# Autodesk Inventor assembly: Weapon Assembly
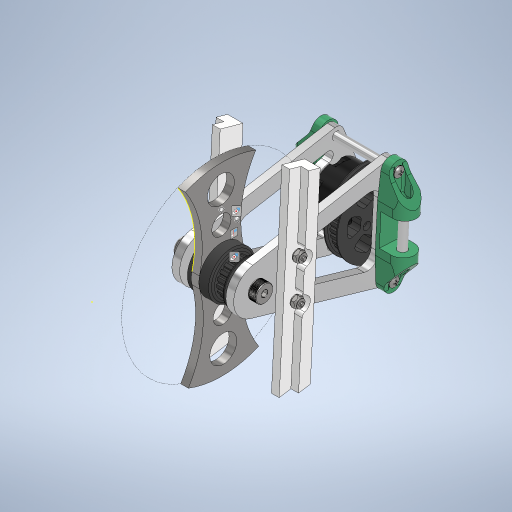
[picture p0: Inventor's stored thumbnail of the model, 512x512]
Saved by Autodesk Inventor 2023.2 (Build 272271000, 271)
## iProperties
Created: 2022-05-21
Part Number: Weapon Assembly
Document SubType Name: Assembly
Designer: Nathan Cai
Mass: 728.967 g
Surface Area: 1305.35 cm^2
Volume: 220.476 cm^3
Density: 3.30633 g/cm^3
Author: Nathan Cai
## Documents named in this file (14)
- E:\Documents\Inventor\0.3rd Lawette - V3.5\Vertical Weapon Assembly (3rd Law)\Weapon Assembly (Vert A).iam
- E:\Documents\Inventor\0.3rd Lawette - V3.5\Standoff 1.5in.ipt
- E:\Documents\Inventor\Content Center Files\R2023\en-US\ANSI B18.6.3(27)\ANSI B18.6.3 - 6-32 UNC - 0.75(11).ipt
- E:\Documents\Inventor\Content Center Files\R2023\en-US\SAE J773b\SAE J773b - No. 6. SAE Type L. narrow.ipt
- E:\Documents\Inventor\Content Center Files\R2023\en-US\IFI 100 107(2)\IFI 100_107 - No. 6 - 32 Metal Type.ipt
- E:\Documents\Inventor\0.3rd Lawette - V3.5\Bracket.ipt
- E:\Documents\Inventor\Content Center Files\R2023\en-US\ANSI B18.6.3(27)\ANSI B18.6.3 - 6-32 UNC - 0.625(11).ipt
- E:\Documents\Inventor\0.3rd Lawette - V3.5\Vertical Weapon Assembly (3rd Law)\Legs.ipt
- E:\Documents\Inventor\0.3rd Lawette - V3.5\Vertical Weapon Assembly (3rd Law)\Frame (Clear Side).ipt
- E:\Documents\Inventor\0.3rd Lawette - V3.5\Vertical Weapon Assembly (3rd Law)\Frame (Motor Side).ipt
- E:\Documents\Inventor\0.3rd Lawette - V3.5\Vertical Weapon Assembly (3rd Law)\90630A121_High-Strength Steel Nylon-Insert Locknut.ipt
- E:\Documents\Inventor\0.3rd Lawette - V3.5\Vertical Weapon Assembly (3rd Law)\90807A139_Same-Size Thread Alloy Steel Shoulder Screw.ipt
- E:\Documents\Inventor\0.3rd Lawette - V3.5\Vertical Weapon Assembly (3rd Law)\Weapon (Motor-Side Pulley).iam
- E:\Documents\Inventor\0.3rd Lawette - V3.5\Vertical Weapon Assembly (3rd Law)\Weapon (Weapon-Side Pulley).iam
## Components (42 placed, 13 different names)
1. Weapon (Weapon-Side Pulley):2 [sub-assembly]
2. Weapon (Motor-Side Pulley):2 [sub-assembly]
3. 90807A139_Same-Size Thread Alloy Steel Shoulder Screw:2
4. 90630A121_High-Strength Steel Nylon-Insert Locknut:2
5. Frame (Motor Side):2
6. Frame (Clear Side):2
7. Legs:3
8. Legs:2 — Mate:231, Mate:233
9. Bracket:1 — Mate:174, Mate:175, Mate:176, Flush:2, Mate:210, Mate:211, Mate:212, Mate:213, Mate:218, Mate:219, Mate:221, Mate:222
10. Bracket:2 — Mate:171, Mate:172, Mate:177, Flush:1, Mate:214, Mate:215, Mate:216, Mate:217, Mate:220, Mate:224
11. Standoff 1.5in:1 — Mate:171, Mate:174
12. Standoff 1.5in:2 — Mate:172, Mate:175
13. Standoff 1.5in:3 — Mate:176, Flush:2, Mate:223, Mate:225
14. Standoff 1.5in:4 — Mate:177, Flush:1
15. Prevailing Torque Type Hex Nut - Inch (IFI) No. 6 - 32 Metal Type:23 — Insert:46
16. Conical Spring Washer SAE J773b (Inch) No. 6. SAE Type L. narrow:39 — Mate:233, Insert:46
17. Cross Recessed Truss Head Machine Screw - Type I - Inch No. 6 - 32 - 3/4:28
18. Prevailing Torque Type Hex Nut - Inch (IFI) No. 6 - 32 Metal Type:19 — Insert:45
19. Conical Spring Washer SAE J773b (Inch) No. 6. SAE Type L. narrow:27 — Mate:231, Insert:45
20. Cross Recessed Truss Head Machine Screw - Type I - Inch No. 6 - 32 - 3/4:20
21. Cross Recessed Truss Head Machine Screw - Type I - Inch No. 6 - 32 - 5/8:8 — Insert:44
22. Conical Spring Washer SAE J773b (Inch) No. 6. SAE Type L. narrow:38 — Mate:224, Mate:225, Insert:44
23. Cross Recessed Truss Head Machine Screw - Type I - Inch No. 6 - 32 - 5/8:7 — Insert:43
24. Conical Spring Washer SAE J773b (Inch) No. 6. SAE Type L. narrow:37 — Mate:222, Mate:223, Insert:43
25. Cross Recessed Truss Head Machine Screw - Type I - Inch No. 6 - 32 - 5/8:6 — Insert:42
26. Conical Spring Washer SAE J773b (Inch) No. 6. SAE Type L. narrow:36 — Mate:220, Mate:221, Insert:42
27. Cross Recessed Truss Head Machine Screw - Type I - Inch No. 6 - 32 - 5/8:5 — Insert:41
28. Conical Spring Washer SAE J773b (Inch) No. 6. SAE Type L. narrow:35 — Mate:218, Mate:219, Insert:41
29. Cross Recessed Truss Head Machine Screw - Type I - Inch No. 6 - 32 - 3/4:27 — Insert:40
30. Conical Spring Washer SAE J773b (Inch) No. 6. SAE Type L. narrow:34 — Mate:216, Mate:217, Insert:40
31. Cross Recessed Truss Head Machine Screw - Type I - Inch No. 6 - 32 - 3/4:26 — Insert:39
32. Conical Spring Washer SAE J773b (Inch) No. 6. SAE Type L. narrow:33 — Mate:214, Mate:215, Insert:39
33. Cross Recessed Truss Head Machine Screw - Type I - Inch No. 6 - 32 - 3/4:25 — Insert:38
34. Conical Spring Washer SAE J773b (Inch) No. 6. SAE Type L. narrow:32 — Mate:212, Mate:213, Insert:38
35. Cross Recessed Truss Head Machine Screw - Type I - Inch No. 6 - 32 - 3/4:24 — Insert:37
36. Conical Spring Washer SAE J773b (Inch) No. 6. SAE Type L. narrow:31 — Mate:210, Mate:211, Insert:37
37. Prevailing Torque Type Hex Nut - Inch (IFI) No. 6 - 32 Metal Type:22 — Insert:36
38. Conical Spring Washer SAE J773b (Inch) No. 6. SAE Type L. narrow:30 — Insert:36
39. Cross Recessed Truss Head Machine Screw - Type I - Inch No. 6 - 32 - 3/4:23
40. Prevailing Torque Type Hex Nut - Inch (IFI) No. 6 - 32 Metal Type:21 — Insert:35
41. Conical Spring Washer SAE J773b (Inch) No. 6. SAE Type L. narrow:29 — Insert:35
42. Cross Recessed Truss Head Machine Screw - Type I - Inch No. 6 - 32 - 3/4:22
## Relationships (77: Mate 62, Insert 12, Flush 2, Symmetry 1)
- [Mate]: 90807A139_Same-Size Thread Alloy Steel Shoulder Screw:2 ↔ 90630A121_High-Strength Steel Nylon-Insert Locknut:2
- [Mate] (50.8 mm): 90807A139_Same-Size Thread Alloy Steel Shoulder Screw:2 ↔ 90630A121_High-Strength Steel Nylon-Insert Locknut:2
- [Mate]: Weapon (Weapon-Side Pulley):2 ↔ 90807A139_Same-Size Thread Alloy Steel Shoulder Screw:2
- [Mate]: 90807A139_Same-Size Thread Alloy Steel Shoulder Screw:2 ↔ Frame (Motor Side):2
- [Mate]: 90807A139_Same-Size Thread Alloy Steel Shoulder Screw:2 ↔ Frame (Clear Side):2
- [Mate]: 90807A139_Same-Size Thread Alloy Steel Shoulder Screw:2 ↔ Frame (Clear Side):2
- [Mate]: Frame (Motor Side):2 ↔ Frame (Clear Side):2
- [Mate]: Frame (Motor Side):2 ↔ Standoff 1.5in:1
- [Mate]: Frame (Motor Side):2 ↔ Standoff 1.5in:2
- [Mate]: Frame (Motor Side):2 ↔ Standoff 1.5in:1
- [Mate]: Frame (Motor Side):2 ↔ Standoff 1.5in:2
- [Mate]: Frame (Clear Side):2 ↔ Legs:3
- [Mate]: Frame (Clear Side):2 ↔ Legs:3
- [Mate]: Frame (Clear Side):2 ↔ Legs:3
- [Mate]: Frame (Clear Side):2 ↔ Standoff 1.5in:1
- [Mate] (0.0254 mm): Weapon (Weapon-Side Pulley):2 ↔ Frame (Motor Side):2
- [Symmetry]: Frame (Motor Side):2 ↔ Frame (Clear Side):2
- [Mate]: Frame (Motor Side):2 ↔ Legs:2
- [Mate]: Frame (Motor Side):2 ↔ Legs:2
- [Mate]: Frame (Motor Side):2 ↔ Legs:2
- [Mate]: Weapon (Motor-Side Pulley):2 ↔ Frame (Motor Side):2
- [Mate]: Weapon (Motor-Side Pulley):2 ↔ Frame (Motor Side):2
- [Mate]: Weapon (Motor-Side Pulley):2 ↔ Frame (Motor Side):2
- [Mate]: Frame (Motor Side):2 ↔ Bracket:2
- Mate:171: Bracket:2 ↔ Standoff 1.5in:1
- Mate:172: Bracket:2 ↔ Standoff 1.5in:2
- [Mate]: Frame (Clear Side):2 ↔ Bracket:1
- Mate:174: Bracket:1 ↔ Standoff 1.5in:1
- Mate:175: Bracket:1 ↔ Standoff 1.5in:2
- Mate:176: Bracket:1 ↔ Standoff 1.5in:3
- Mate:177: Bracket:2 ↔ Standoff 1.5in:4
- Flush:1: Bracket:2 ↔ Standoff 1.5in:4
- Flush:2: Bracket:1 ↔ Standoff 1.5in:3
- [Mate]: Frame (Clear Side):2 ↔ Cross Recessed Truss Head Machine Screw - Type I - Inch No. 6 - 32 - 3/4:22
- [Mate]: Frame (Clear Side):2 ↔ Cross Recessed Truss Head Machine Screw - Type I - Inch No. 6 - 32 - 3/4:22
- [Mate]: Frame (Clear Side):2 ↔ Cross Recessed Truss Head Machine Screw - Type I - Inch No. 6 - 32 - 3/4:23
- [Mate]: Frame (Clear Side):2 ↔ Cross Recessed Truss Head Machine Screw - Type I - Inch No. 6 - 32 - 3/4:23
- [Mate]: Frame (Clear Side):2 ↔ Conical Spring Washer SAE J773b (Inch) No. 6. SAE Type L. narrow:29
- [Mate]: Legs:3 ↔ Conical Spring Washer SAE J773b (Inch) No. 6. SAE Type L. narrow:29
- [Mate]: Frame (Clear Side):2 ↔ Conical Spring Washer SAE J773b (Inch) No. 6. SAE Type L. narrow:30
- [Mate]: Legs:3 ↔ Conical Spring Washer SAE J773b (Inch) No. 6. SAE Type L. narrow:30
- Insert:35: Prevailing Torque Type Hex Nut - Inch (IFI) No. 6 - 32 Metal Type:21 ↔ Conical Spring Washer SAE J773b (Inch) No. 6. SAE Type L. narrow:29
- Insert:36: Prevailing Torque Type Hex Nut - Inch (IFI) No. 6 - 32 Metal Type:22 ↔ Conical Spring Washer SAE J773b (Inch) No. 6. SAE Type L. narrow:30
- Mate:210: Bracket:1 ↔ Conical Spring Washer SAE J773b (Inch) No. 6. SAE Type L. narrow:31
- Mate:211: Bracket:1 ↔ Conical Spring Washer SAE J773b (Inch) No. 6. SAE Type L. narrow:31
- Mate:212: Bracket:1 ↔ Conical Spring Washer SAE J773b (Inch) No. 6. SAE Type L. narrow:32
- Mate:213: Bracket:1 ↔ Conical Spring Washer SAE J773b (Inch) No. 6. SAE Type L. narrow:32
- Insert:37: Cross Recessed Truss Head Machine Screw - Type I - Inch No. 6 - 32 - 3/4:24 ↔ Conical Spring Washer SAE J773b (Inch) No. 6. SAE Type L. narrow:31
- Insert:38: Cross Recessed Truss Head Machine Screw - Type I - Inch No. 6 - 32 - 3/4:25 ↔ Conical Spring Washer SAE J773b (Inch) No. 6. SAE Type L. narrow:32
- Mate:214: Bracket:2 ↔ Conical Spring Washer SAE J773b (Inch) No. 6. SAE Type L. narrow:33
- Mate:215: Bracket:2 ↔ Conical Spring Washer SAE J773b (Inch) No. 6. SAE Type L. narrow:33
- Mate:216: Bracket:2 ↔ Conical Spring Washer SAE J773b (Inch) No. 6. SAE Type L. narrow:34
- Mate:217: Bracket:2 ↔ Conical Spring Washer SAE J773b (Inch) No. 6. SAE Type L. narrow:34
- Insert:39: Cross Recessed Truss Head Machine Screw - Type I - Inch No. 6 - 32 - 3/4:26 ↔ Conical Spring Washer SAE J773b (Inch) No. 6. SAE Type L. narrow:33
- Insert:40: Cross Recessed Truss Head Machine Screw - Type I - Inch No. 6 - 32 - 3/4:27 ↔ Conical Spring Washer SAE J773b (Inch) No. 6. SAE Type L. narrow:34
- Mate:218: Bracket:1 ↔ Conical Spring Washer SAE J773b (Inch) No. 6. SAE Type L. narrow:35
- Mate:219: Bracket:1 ↔ Conical Spring Washer SAE J773b (Inch) No. 6. SAE Type L. narrow:35
- Mate:220: Bracket:2 ↔ Conical Spring Washer SAE J773b (Inch) No. 6. SAE Type L. narrow:36
- Mate:221: Bracket:1 ↔ Conical Spring Washer SAE J773b (Inch) No. 6. SAE Type L. narrow:36
- Insert:41: Cross Recessed Truss Head Machine Screw - Type I - Inch No. 6 - 32 - 5/8:5 ↔ Conical Spring Washer SAE J773b (Inch) No. 6. SAE Type L. narrow:35
- Insert:42: Cross Recessed Truss Head Machine Screw - Type I - Inch No. 6 - 32 - 5/8:6 ↔ Conical Spring Washer SAE J773b (Inch) No. 6. SAE Type L. narrow:36
- Mate:222: Bracket:1 ↔ Conical Spring Washer SAE J773b (Inch) No. 6. SAE Type L. narrow:37
- Mate:223: Standoff 1.5in:3 ↔ Conical Spring Washer SAE J773b (Inch) No. 6. SAE Type L. narrow:37
- Mate:224: Bracket:2 ↔ Conical Spring Washer SAE J773b (Inch) No. 6. SAE Type L. narrow:38
- Mate:225: Standoff 1.5in:3 ↔ Conical Spring Washer SAE J773b (Inch) No. 6. SAE Type L. narrow:38
- Insert:43: Cross Recessed Truss Head Machine Screw - Type I - Inch No. 6 - 32 - 5/8:7 ↔ Conical Spring Washer SAE J773b (Inch) No. 6. SAE Type L. narrow:37
- Insert:44: Cross Recessed Truss Head Machine Screw - Type I - Inch No. 6 - 32 - 5/8:8 ↔ Conical Spring Washer SAE J773b (Inch) No. 6. SAE Type L. narrow:38
- [Mate]: Frame (Motor Side):2 ↔ Cross Recessed Truss Head Machine Screw - Type I - Inch No. 6 - 32 - 3/4:20
- [Mate]: Frame (Motor Side):2 ↔ Cross Recessed Truss Head Machine Screw - Type I - Inch No. 6 - 32 - 3/4:20
- [Mate]: Frame (Motor Side):2 ↔ Cross Recessed Truss Head Machine Screw - Type I - Inch No. 6 - 32 - 3/4:28
- [Mate]: Frame (Motor Side):2 ↔ Cross Recessed Truss Head Machine Screw - Type I - Inch No. 6 - 32 - 3/4:28
- [Mate]: Frame (Motor Side):2 ↔ Conical Spring Washer SAE J773b (Inch) No. 6. SAE Type L. narrow:27
- Mate:231: Legs:2 ↔ Conical Spring Washer SAE J773b (Inch) No. 6. SAE Type L. narrow:27
- [Mate]: Frame (Motor Side):2 ↔ Conical Spring Washer SAE J773b (Inch) No. 6. SAE Type L. narrow:39
- Mate:233: Legs:2 ↔ Conical Spring Washer SAE J773b (Inch) No. 6. SAE Type L. narrow:39
- Insert:45: Prevailing Torque Type Hex Nut - Inch (IFI) No. 6 - 32 Metal Type:19 ↔ Conical Spring Washer SAE J773b (Inch) No. 6. SAE Type L. narrow:27
- Insert:46: Prevailing Torque Type Hex Nut - Inch (IFI) No. 6 - 32 Metal Type:23 ↔ Conical Spring Washer SAE J773b (Inch) No. 6. SAE Type L. narrow:39
